# Autodesk Inventor assembly: 6P Sprocket
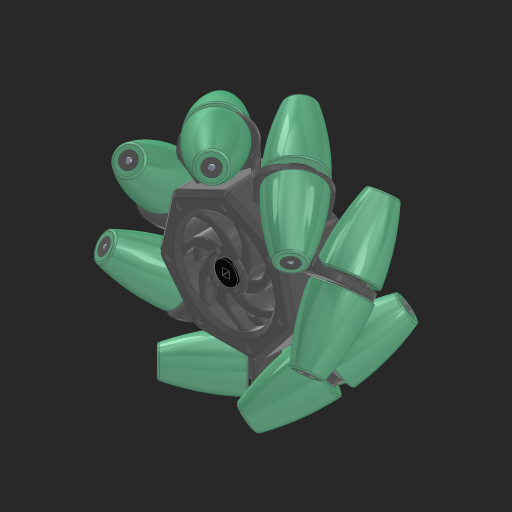
[picture p0: Inventor's stored thumbnail of the model, 512x512]
Saved by Autodesk Inventor 2023 (Build 270158000, 158)
## iProperties
Created: 2022-08-02
Part Number: 6P Sprocket
Document SubType Name: Assembly
Designer: ylu12
Author: ylu12
## Documents named in this file (4)
- C:\Users\ylu12\Documents\GitHub\VEX-CAD-Inventor\Motion\Wheels\Mecanum Wheel\4 Mecanum Right, Square.iam
- C:\Users\ylu12\Documents\GitHub\VEX-CAD-Inventor\Motion\Insert Square.ipt
- C:\Users\ylu12\Documents\GitHub\VEX-CAD-Inventor\Motion\Wheels\Reference Files\4 Mecanum Right.ipt
- C:\Users\ylu12\Documents\GitHub\VEX-CAD-Inventor\Motion\Wheels\Mecanum Wheel.iam
## Components (3 placed, 3 different names)
1. 4 Mecanum Right:1
2. Square 1 — Mate:28, Angle:2, Symmetry:1
3. Square 2 — Mate:27, Angle:1, Symmetry:1, Flush:12
## Relationships (9: Mate 4, Flush 2, Angle 2, Symmetry 1)
- [Flush]: 4 Mecanum Right:1
- [Mate]: 4 Mecanum Right:1
- [Mate]: 4 Mecanum Right:1
- Mate:27: Square 2
- Mate:28: Square 1
- Angle:1 (0 deg): Square 2
- Angle:2 (0 deg): Square 1
- Symmetry:1: Square 1 ↔ Square 2
- Flush:12 (12 mm): Square 2
## Named parameters: Thickness = 12 mm
